# Autodesk Inventor assembly: FullBottom
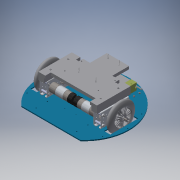
[picture p0: Inventor's stored thumbnail of the model, 180x180]
Saved by Autodesk Inventor 2019 (Build 230136000, 136)
## iProperties
Created: 2019-09-28
Part Number: FullBottom
Document SubType Name: Assembly
Designer: james
Author: james
## Documents named in this file (11)
- F:\JimsDesign\Jims2020FTC\FullBottom.iam
- F:\JimsDesign\Jims2020FTC\BottomPlate.ipt
- F:\JimsDesign\Library\AndyMark\am-3448 PicoBox Duo REV2.iam
- F:\JimsDesign\Jims2020FTC\FullWheel.iam
- F:\JimsDesign\Jims2020FTC\BatteryRail.ipt
- F:\JimsDesign\Library\RevRobotics\REV-31-1302.ipt
- F:\JimsDesign\Jims2020FTC\Slider.ipt
- F:\JimsDesign\Library\McMaster\SocketScrews\91251A197_BLACK-OXIDE ALLOY STEEL SOCKET HEAD CAP SCREW.ipt
- F:\JimsDesign\Jims2020FTC\MotorPlate.ipt
- F:\JimsDesign\Library\McMaster\SocketScrews\91251A201_BLACK-OXIDE ALLOY STEEL SOCKET HEAD SCREW.ipt
- F:\JimsDesign\Library\McMaster\SocketScrews\91251A194_BLACK-OXIDE ALLOY STEEL SOCKET HEAD CAP SCREW.ipt
## Components (35 placed, 10 different names)
1. BottomPlate:1 — Mate:1, Mate:2, Mate:3, Mate:4, Mate:8, Mate:9, Mate:10, Mate:11, Mate:12, Mate:13, Mate:20, Mate:21, Mate:27, Mate:28, Mate:29, Mate:30, Mate:31, Mate:32, Mate:33, Mate:34, Mate:35, Mate:36, Mate:37, Mate:38, Mate:39, Mate:40, Mate:41, Mate:42, Mate:43, Mate:44, Mate:45, Mate:46, Mate:47, Mate:48, Mate:61, Mate:62, Mate:63, Mate:64, Mate:65, Mate:66, Mate:67, Mate:68, Mate:69, Mate:70, Mate:71, Mate:72, Mate:73, Mate:74, Mate:75, Mate:76
2. am-3448 PicoBox Duo REV2:1 [sub-assembly] — Mate:2, Mate:4, Mate:6, Mate:21, Mate:50, Mate:52, Mate:86
3. am-3448 PicoBox Duo REV2:2 [sub-assembly] — Mate:1, Mate:3, Mate:20, Mate:22, Mate:51, Mate:85
4. FullWheel:1 [sub-assembly] — Mate:6, Mate:86
5. FullWheel:2 [sub-assembly] — Mate:22, Mate:85
6. BatteryRail:1 — Mate:8, Mate:9, Mate:10, Mate:15, Mate:49
7. BatteryRail:2 — Mate:11, Mate:12, Mate:13
8. REV-31-1302:1 — Mate:15, Mate:49
9. Slider:1 — Mate:27, Mate:29, Mate:30
10. Slider:2 — Mate:28, Mate:31, Mate:32
11. 91251A197_BLACK-OXIDE ALLOY STEEL SOCKET HEAD CAP SCREW:1 — Mate:34, Mate:36
12. 91251A197_BLACK-OXIDE ALLOY STEEL SOCKET HEAD CAP SCREW:2 — Mate:33, Mate:35
13. 91251A197_BLACK-OXIDE ALLOY STEEL SOCKET HEAD CAP SCREW:3 — Mate:41, Mate:43
14. 91251A197_BLACK-OXIDE ALLOY STEEL SOCKET HEAD CAP SCREW:4 — Mate:42, Mate:44
15. 91251A197_BLACK-OXIDE ALLOY STEEL SOCKET HEAD CAP SCREW:5 — Mate:46, Mate:48
16. 91251A197_BLACK-OXIDE ALLOY STEEL SOCKET HEAD CAP SCREW:6 — Mate:45, Mate:47
17. 91251A197_BLACK-OXIDE ALLOY STEEL SOCKET HEAD CAP SCREW:7 — Mate:38, Mate:39
18. 91251A197_BLACK-OXIDE ALLOY STEEL SOCKET HEAD CAP SCREW:8 — Mate:37, Mate:40
19. MotorPlate:1 — Mate:50, Mate:51, Mate:52, Mate:53, Mate:54, Mate:55, Mate:56, Mate:57, Mate:58, Mate:59, Mate:60, Mate:77, Mate:78, Mate:79, Mate:80, Mate:81, Mate:82, Mate:83, Mate:84
20. 91251A201_BLACK-OXIDE ALLOY STEEL SOCKET HEAD SCREW:1 — Mate:56, Mate:59
21. 91251A201_BLACK-OXIDE ALLOY STEEL SOCKET HEAD SCREW:2 — Mate:55, Mate:60
22. 91251A201_BLACK-OXIDE ALLOY STEEL SOCKET HEAD SCREW:3 — Mate:54, Mate:57
23. 91251A201_BLACK-OXIDE ALLOY STEEL SOCKET HEAD SCREW:4 — Mate:53, Mate:58
24. 91251A194_BLACK-OXIDE ALLOY STEEL SOCKET HEAD CAP SCREW:1 — Mate:61, Mate:71
25. 91251A194_BLACK-OXIDE ALLOY STEEL SOCKET HEAD CAP SCREW:2 — Mate:62, Mate:75
26. 91251A194_BLACK-OXIDE ALLOY STEEL SOCKET HEAD CAP SCREW:3 — Mate:64, Mate:72
27. 91251A194_BLACK-OXIDE ALLOY STEEL SOCKET HEAD CAP SCREW:4 — Mate:65, Mate:73
28. 91251A194_BLACK-OXIDE ALLOY STEEL SOCKET HEAD CAP SCREW:5 — Mate:63, Mate:74
29. 91251A194_BLACK-OXIDE ALLOY STEEL SOCKET HEAD CAP SCREW:6 — Mate:66, Mate:76
30. 91251A194_BLACK-OXIDE ALLOY STEEL SOCKET HEAD CAP SCREW:7 — Mate:67, Mate:70
31. 91251A194_BLACK-OXIDE ALLOY STEEL SOCKET HEAD CAP SCREW:8 — Mate:68, Mate:69
32. 91251A201_BLACK-OXIDE ALLOY STEEL SOCKET HEAD SCREW:5 — Mate:80, Mate:82
33. 91251A201_BLACK-OXIDE ALLOY STEEL SOCKET HEAD SCREW:6 — Mate:79, Mate:83
34. 91251A201_BLACK-OXIDE ALLOY STEEL SOCKET HEAD SCREW:7 — Mate:78, Mate:84
35. 91251A201_BLACK-OXIDE ALLOY STEEL SOCKET HEAD SCREW:8 — Mate:77, Mate:81
## Relationships (75: Mate 75)
- Mate:1: BottomPlate:1 ↔ am-3448 PicoBox Duo REV2:2
- Mate:2: BottomPlate:1 ↔ am-3448 PicoBox Duo REV2:1
- Mate:3: BottomPlate:1 ↔ am-3448 PicoBox Duo REV2:2
- Mate:4: BottomPlate:1 ↔ am-3448 PicoBox Duo REV2:1
- Mate:6: am-3448 PicoBox Duo REV2:1 ↔ FullWheel:1
- Mate:8: BottomPlate:1 ↔ BatteryRail:1
- Mate:9: BottomPlate:1 ↔ BatteryRail:1
- Mate:10: BottomPlate:1 ↔ BatteryRail:1
- Mate:11: BottomPlate:1 ↔ BatteryRail:2
- Mate:12: BottomPlate:1 ↔ BatteryRail:2
- Mate:13: BottomPlate:1 ↔ BatteryRail:2
- Mate:15: BatteryRail:1 ↔ REV-31-1302:1
- Mate:20: BottomPlate:1 ↔ am-3448 PicoBox Duo REV2:2
- Mate:21: BottomPlate:1 ↔ am-3448 PicoBox Duo REV2:1
- Mate:22: am-3448 PicoBox Duo REV2:2 ↔ FullWheel:2
- Mate:27: BottomPlate:1 ↔ Slider:1
- Mate:28: BottomPlate:1 ↔ Slider:2
- Mate:29: BottomPlate:1 ↔ Slider:1
- Mate:30: BottomPlate:1 ↔ Slider:1
- Mate:31: BottomPlate:1 ↔ Slider:2
- Mate:32: BottomPlate:1 ↔ Slider:2
- Mate:33: BottomPlate:1 ↔ 91251A197_BLACK-OXIDE ALLOY STEEL SOCKET HEAD CAP SCREW:2
- Mate:34: BottomPlate:1 ↔ 91251A197_BLACK-OXIDE ALLOY STEEL SOCKET HEAD CAP SCREW:1
- Mate:35: BottomPlate:1 ↔ 91251A197_BLACK-OXIDE ALLOY STEEL SOCKET HEAD CAP SCREW:2
- Mate:36: BottomPlate:1 ↔ 91251A197_BLACK-OXIDE ALLOY STEEL SOCKET HEAD CAP SCREW:1
- Mate:37: BottomPlate:1 ↔ 91251A197_BLACK-OXIDE ALLOY STEEL SOCKET HEAD CAP SCREW:8
- Mate:38: BottomPlate:1 ↔ 91251A197_BLACK-OXIDE ALLOY STEEL SOCKET HEAD CAP SCREW:7
- Mate:39: BottomPlate:1 ↔ 91251A197_BLACK-OXIDE ALLOY STEEL SOCKET HEAD CAP SCREW:7
- Mate:40: BottomPlate:1 ↔ 91251A197_BLACK-OXIDE ALLOY STEEL SOCKET HEAD CAP SCREW:8
- Mate:41: BottomPlate:1 ↔ 91251A197_BLACK-OXIDE ALLOY STEEL SOCKET HEAD CAP SCREW:3
- Mate:42: BottomPlate:1 ↔ 91251A197_BLACK-OXIDE ALLOY STEEL SOCKET HEAD CAP SCREW:4
- Mate:43: BottomPlate:1 ↔ 91251A197_BLACK-OXIDE ALLOY STEEL SOCKET HEAD CAP SCREW:3
- Mate:44: BottomPlate:1 ↔ 91251A197_BLACK-OXIDE ALLOY STEEL SOCKET HEAD CAP SCREW:4
- Mate:45: BottomPlate:1 ↔ 91251A197_BLACK-OXIDE ALLOY STEEL SOCKET HEAD CAP SCREW:6
- Mate:46: BottomPlate:1 ↔ 91251A197_BLACK-OXIDE ALLOY STEEL SOCKET HEAD CAP SCREW:5
- Mate:47: BottomPlate:1 ↔ 91251A197_BLACK-OXIDE ALLOY STEEL SOCKET HEAD CAP SCREW:6
- Mate:48: BottomPlate:1 ↔ 91251A197_BLACK-OXIDE ALLOY STEEL SOCKET HEAD CAP SCREW:5
- Mate:49: BatteryRail:1 ↔ REV-31-1302:1
- Mate:50: am-3448 PicoBox Duo REV2:1 ↔ MotorPlate:1
- Mate:51: am-3448 PicoBox Duo REV2:2 ↔ MotorPlate:1
- Mate:52: am-3448 PicoBox Duo REV2:1 ↔ MotorPlate:1
- Mate:53: MotorPlate:1 ↔ 91251A201_BLACK-OXIDE ALLOY STEEL SOCKET HEAD SCREW:4
- Mate:54: MotorPlate:1 ↔ 91251A201_BLACK-OXIDE ALLOY STEEL SOCKET HEAD SCREW:3
- Mate:55: MotorPlate:1 ↔ 91251A201_BLACK-OXIDE ALLOY STEEL SOCKET HEAD SCREW:2
- Mate:56: MotorPlate:1 ↔ 91251A201_BLACK-OXIDE ALLOY STEEL SOCKET HEAD SCREW:1
- Mate:57: MotorPlate:1 ↔ 91251A201_BLACK-OXIDE ALLOY STEEL SOCKET HEAD SCREW:3
- Mate:58: MotorPlate:1 ↔ 91251A201_BLACK-OXIDE ALLOY STEEL SOCKET HEAD SCREW:4
- Mate:59: MotorPlate:1 ↔ 91251A201_BLACK-OXIDE ALLOY STEEL SOCKET HEAD SCREW:1
- Mate:60: MotorPlate:1 ↔ 91251A201_BLACK-OXIDE ALLOY STEEL SOCKET HEAD SCREW:2
- Mate:61: BottomPlate:1 ↔ 91251A194_BLACK-OXIDE ALLOY STEEL SOCKET HEAD CAP SCREW:1
- Mate:62: BottomPlate:1 ↔ 91251A194_BLACK-OXIDE ALLOY STEEL SOCKET HEAD CAP SCREW:2
- Mate:63: BottomPlate:1 ↔ 91251A194_BLACK-OXIDE ALLOY STEEL SOCKET HEAD CAP SCREW:5
- Mate:64: BottomPlate:1 ↔ 91251A194_BLACK-OXIDE ALLOY STEEL SOCKET HEAD CAP SCREW:3
- Mate:65: BottomPlate:1 ↔ 91251A194_BLACK-OXIDE ALLOY STEEL SOCKET HEAD CAP SCREW:4
- Mate:66: BottomPlate:1 ↔ 91251A194_BLACK-OXIDE ALLOY STEEL SOCKET HEAD CAP SCREW:6
- Mate:67: BottomPlate:1 ↔ 91251A194_BLACK-OXIDE ALLOY STEEL SOCKET HEAD CAP SCREW:7
- Mate:68: BottomPlate:1 ↔ 91251A194_BLACK-OXIDE ALLOY STEEL SOCKET HEAD CAP SCREW:8
- Mate:69: BottomPlate:1 ↔ 91251A194_BLACK-OXIDE ALLOY STEEL SOCKET HEAD CAP SCREW:8
- Mate:70: BottomPlate:1 ↔ 91251A194_BLACK-OXIDE ALLOY STEEL SOCKET HEAD CAP SCREW:7
- Mate:71: BottomPlate:1 ↔ 91251A194_BLACK-OXIDE ALLOY STEEL SOCKET HEAD CAP SCREW:1
- Mate:72: BottomPlate:1 ↔ 91251A194_BLACK-OXIDE ALLOY STEEL SOCKET HEAD CAP SCREW:3
- Mate:73: BottomPlate:1 ↔ 91251A194_BLACK-OXIDE ALLOY STEEL SOCKET HEAD CAP SCREW:4
- Mate:74: BottomPlate:1 ↔ 91251A194_BLACK-OXIDE ALLOY STEEL SOCKET HEAD CAP SCREW:5
- Mate:75: BottomPlate:1 ↔ 91251A194_BLACK-OXIDE ALLOY STEEL SOCKET HEAD CAP SCREW:2
- Mate:76: BottomPlate:1 ↔ 91251A194_BLACK-OXIDE ALLOY STEEL SOCKET HEAD CAP SCREW:6
- Mate:77: MotorPlate:1 ↔ 91251A201_BLACK-OXIDE ALLOY STEEL SOCKET HEAD SCREW:8
- Mate:78: MotorPlate:1 ↔ 91251A201_BLACK-OXIDE ALLOY STEEL SOCKET HEAD SCREW:7
- Mate:79: MotorPlate:1 ↔ 91251A201_BLACK-OXIDE ALLOY STEEL SOCKET HEAD SCREW:6
- Mate:80: MotorPlate:1 ↔ 91251A201_BLACK-OXIDE ALLOY STEEL SOCKET HEAD SCREW:5
- Mate:81: MotorPlate:1 ↔ 91251A201_BLACK-OXIDE ALLOY STEEL SOCKET HEAD SCREW:8
- Mate:82: MotorPlate:1 ↔ 91251A201_BLACK-OXIDE ALLOY STEEL SOCKET HEAD SCREW:5
- Mate:83: MotorPlate:1 ↔ 91251A201_BLACK-OXIDE ALLOY STEEL SOCKET HEAD SCREW:6
- Mate:84: MotorPlate:1 ↔ 91251A201_BLACK-OXIDE ALLOY STEEL SOCKET HEAD SCREW:7
- Mate:85: am-3448 PicoBox Duo REV2:2 ↔ FullWheel:2
- Mate:86: am-3448 PicoBox Duo REV2:1 ↔ FullWheel:1
